# Autodesk Inventor assembly: PhoneCordHolder
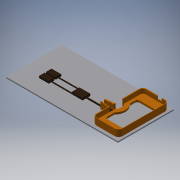
[picture p0: Inventor's stored thumbnail of the model, 180x180]
Saved by Autodesk Inventor 2017 (Build 210142000, 142)
## iProperties
Created: 2017-12-02
Part Number: PhoneCordHolder
Document SubType Name: Assembly
Designer: User
Author: User
## Documents named in this file (4)
- C:\Robotics\CAD\2017-18_CAD\PhoneCordHolder.iam
- C:\Robotics\CAD\2017-18_CAD\phone holder base.ipt
- C:\Robotics\CAD\2017-18_CAD\Phone_Case_Driver.ipt
- C:\Robotics\CAD\2017-18_CAD\phone wire.ipt
## Components (3 placed, 3 different names)
1. phone holder base:1 — Mate:1, Flush:1, Flush:2, Mate:2
2. Phone_Case_Driver:1 — Mate:1, Flush:1, Flush:2, Flush:3, Mate:3
3. phone wire:1 — Mate:2, Flush:3, Mate:3
## Relationships (6: Mate 3, Flush 3)
- Mate:1: phone holder base:1 ↔ Phone_Case_Driver:1
- Flush:1 (6.35 mm): phone holder base:1 ↔ Phone_Case_Driver:1
- Flush:2 (6.35 mm): phone holder base:1 ↔ Phone_Case_Driver:1
- Mate:2: phone holder base:1 ↔ phone wire:1
- Flush:3: Phone_Case_Driver:1 ↔ phone wire:1
- Mate:3: Phone_Case_Driver:1 ↔ phone wire:1
